# Autodesk Inventor assembly: GP7-100
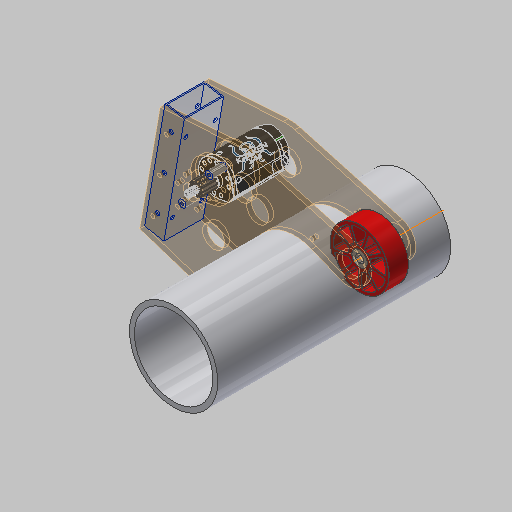
[picture p0: Inventor's stored thumbnail of the model, 512x512]
Saved by Autodesk Inventor 2023.5 (Build 275446000, 446)
## iProperties
Created: 2025-02-24
Part Number: GP7-100
Document SubType Name: Assembly
Designer: dlangdon
Author: dlangdon
## Documents named in this file (11)
- C:\Users\slick\OneDrive\Desktop\2025-ReefScape---CAD\Gripper\GP7\GP7-100.iam
- C:\Users\slick\OneDrive\Desktop\2025-ReefScape---CAD\Gripper\GP7\GP7-001.ipt
- C:\Users\slick\OneDrive\Desktop\2025-ReefScape---CAD\Gripper\GP7\GP7-003.ipt
- C:\Users\slick\OneDrive\Desktop\2025-ReefScape---CAD\COMMON PARTS\MOTORS\WCP-0941 x44 Kracken.ipt
- C:\Users\slick\OneDrive\Desktop\2025-ReefScape---CAD\COMMON PARTS\GEARS\12t 20 dp kracken WCP-1010.ipt
- C:\Users\slick\OneDrive\Desktop\2025-ReefScape---CAD\Gripper\GP6\GP6-006.ipt
- C:\Users\slick\OneDrive\Desktop\2025-ReefScape---CAD\Gripper\GP7\GP7-004.ipt
- C:\Users\slick\OneDrive\Desktop\2025-ReefScape---CAD\Gripper\GP7\GP7-002.ipt
- C:\Users\slick\OneDrive\Desktop\2025-ReefScape---CAD\COMMON PARTS\WHEELS\am-3946 3IN 375Hex Compliant Wheel REV 3.ipt
- C:\Users\slick\OneDrive\Desktop\2025-ReefScape---CAD\COMMON PARTS\WHEELS\Andymark 2 in Wheelam-3155 2IN 500Hex Stealth Wheel REV2.iam
- C:\Users\slick\OneDrive\Desktop\2025-ReefScape---CAD\Field Items\Game Pieces\GE-25500.ipt
## Components (11 placed, 10 different names)
1. GP7-001:1 — Insert:6, Insert:7, Insert:8, Insert:9, Mate:2, Tangent:2, Mate:3
2. GP7-003:1 — Insert:1, Insert:2, Insert:4, Insert:5
3. WCP-0941 x44 Kracken:1 — Insert:1, Insert:2, Insert:3
4. 12t 20 dp kracken WCP-1010:1 — Insert:3
5. GP6-006:1 — Insert:5, Insert:7
6. GP6-006:2 — Insert:4, Insert:6
7. GP7-004:1 — Insert:8, Insert:9, Insert:10, Insert:11
8. GP7-002:1 — Insert:10, Insert:11, Mate:1, Tangent:1
9. am-3946 3IN 375Hex Compliant Wheel REV 3:1 — Mate:1
10. Andymark 2 in Wheelam-3155 2IN 500Hex Stealth Wheel REV2:1 [sub-assembly] — Mate:2
11. GE-25500:1 — Tangent:1, Tangent:2, Mate:3
## Relationships (16: Insert 11, Mate 3, Tangent 2)
- Insert:1: GP7-003:1 ↔ WCP-0941 x44 Kracken:1
- Insert:2: GP7-003:1 ↔ WCP-0941 x44 Kracken:1
- Insert:3: WCP-0941 x44 Kracken:1 ↔ 12t 20 dp kracken WCP-1010:1
- Insert:4: GP7-003:1 ↔ GP6-006:2
- Insert:5: GP7-003:1 ↔ GP6-006:1
- Insert:6: GP7-001:1 ↔ GP6-006:2
- Insert:7: GP7-001:1 ↔ GP6-006:1
- Insert:8: GP7-001:1 ↔ GP7-004:1
- Insert:9: GP7-001:1 ↔ GP7-004:1
- Insert:10: GP7-004:1 ↔ GP7-002:1
- Insert:11: GP7-004:1 ↔ GP7-002:1
- Mate:1: GP7-002:1 ↔ am-3946 3IN 375Hex Compliant Wheel REV 3:1
- Mate:2: GP7-001:1 ↔ Andymark 2 in Wheelam-3155 2IN 500Hex Stealth Wheel REV2:1
- Tangent:1: GP7-002:1 ↔ GE-25500:1
- Tangent:2: GP7-001:1 ↔ GE-25500:1
- Mate:3: GP7-001:1 ↔ GE-25500:1
